# Autodesk Inventor assembly: Assembly3
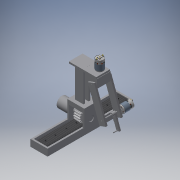
[picture p0: Inventor's stored thumbnail of the model, 180x180]
Saved by Autodesk Inventor 2019.4 (Build 234330000, 330)
## iProperties
Created: 2020-04-15
Part Number: Assembly3
Document SubType Name: Assembly
Designer: Niran
Author: Niran
## iProperties of the stored document S.gear.ipt
Created: 2020-04-14
Part Number: S.gear
Material: Generic
Document SubType Name: Modeling
Designer: Darugar
Density: 1 g/cm^3
Appearance: Default
Author: Darugar
Sending System: Autodesk Inventor 2020
## iProperties of the stored document S.motor.ipt
Created: 2020-04-14
Part Number: S.motor
Material: Generic
Document SubType Name: Modeling
Designer: Darugar
Density: 1 g/cm^3
Appearance: Default
Author: Darugar
Sending System: Autodesk Inventor 2020
## iProperties of the stored document S.Platform.ipt
Created: 2020-04-14
Part Number: S.Platform
Material: Generic
Document SubType Name: Modeling
Designer: Darugar
Density: 1 g/cm^3
Appearance: Default
Author: Darugar
Sending System: Autodesk Inventor 2020
## iProperties of the stored document s.Strikrt.ipt
Created: 2020-04-14
Part Number: s.Strikrt
Material: Generic
Document SubType Name: Modeling
Designer: Darugar
Density: 1 g/cm^3
Appearance: Default
Author: Darugar
Sending System: Autodesk Inventor 2020
## iProperties of the stored document S.rack.ipt
Created: 2020-04-14
Part Number: S.rack
Material: Generic
Document SubType Name: Modeling
Designer: Darugar
Density: 1 g/cm^3
Appearance: Default
Author: Darugar
Sending System: Autodesk Inventor 2020
## iProperties of the stored document S.hollow box.ipt
Created: 2020-04-13
Part Number: S.hollow box
Material: Generic
Document SubType Name: Modeling
Designer: Darugar
Density: 1 g/cm^3
Appearance: Default
Author: Darugar
Sending System: Autodesk Inventor 2020
## Documents named in this file (20)
- **C:\Users\Niran\Desktop\S.Carrom_bot\Assembly3.iam*LocalDocs*xDrle05f4Rw1buugfIqzzd3tlMb*S.gear.ipt
- **C:\Users\Niran\Desktop\S.Carrom_bot\Assembly3.iam*LocalDocs*x122kn5ufNzxlefwdNu51dwe40f*S.motor.ipt
- **C:\Users\Niran\Desktop\S.Carrom_bot\Assembly3.iam*LocalDocs*x0acgfz2z0tlie3kiGyxgdtb3Ig*S.Platform.ipt
- **C:\Users\Niran\Desktop\S.Carrom_bot\Assembly3.iam*LocalDocs*xOnqyxwphSiaaenkcZqvwvmabYh*s.Strikrt.ipt
- **C:\Users\Niran\Desktop\S.Carrom_bot\Assembly3.iam*LocalDocs*xMjvgupfc2g05uukt4i5agsne0h*S.rack.ipt
- **C:\Users\Niran\Desktop\S.Carrom_bot\Assembly3.iam*LocalDocs*xZqkpyfp0KfdfunouZc1cgw1dQb*S.hollow box.ipt
- C:\Users\Niran\Desktop\S.Carrom_bot\Assembly3.iam
- C:\Users\Niran\Desktop\S.Carrom_bot\S.Part1143.ipt
- C:\Users\Niran\Desktop\S.Carrom_bot\DC Motor.ipt
- C:\Users\Niran\Desktop\sketch_jan26a\Canon parts\Part36.ipt
- C:\Users\Niran\Desktop\S.Carrom_bot\Part59.ipt
- C:\Users\Niran\Desktop\S.Carrom_bot\Part13.ipt
- C:\Users\Niran\Desktop\S.Carrom_bot\Part14.ipt
- C:\Users\Niran\Desktop\sketch_jan26a\Canon parts\DC Motor.ipt
- C:\Users\Niran\Desktop\S.Carrom_bot\S.hollow box.ipt
- C:\Users\Niran\Desktop\S.Carrom_bot\S.rack.ipt
- C:\Users\Niran\Desktop\S.Carrom_bot\S.Platform.ipt
- C:\Users\Niran\Desktop\S.Carrom_bot\S.motor.ipt
- C:\Users\Niran\Desktop\S.Carrom_bot\S.gear.ipt
- C:\Users\Niran\Desktop\S.Carrom_bot\s.Strikrt.ipt
## Components (16 placed, 12 different names)
1. S.hollow box:1 — Rotational:1, Rotational:2
2. S.rack:1 — Rotational:1
3. S.Platform:1 — Rotational:2, Rotational:3, Rigid:3
4. S.motor:1 — Rotational:3, Rigid:1
5. S.gear:1 — Rigid:1
6. S.Part1143:1 — Rigid:2, Rigid:3
7. S.Part1143:2 — Rigid:2, Rigid:4, Rotational:4, Rotational:5
8. DC Motor:1 — Rigid:4
9. Part59:1 — Rotational:4
10. Part13:1 — Rotational:5, Rotational:6, Rotational:7
11. Part14:1 — Rotational:6, Rotational:8
12. Part14:2 — Rotational:7
13. Part36:1 — Rotational:8, Rotational:9, Rotational:10, Rigid:5
14. Part36:3 — Rotational:10
15. s.Strikrt:1 — Rotational:9
16. DC Motor:2 — Rigid:5
## Relationships (15: RevoluteJoint 10, WeldJoint 5)
- Rotational:1 [RevoluteJoint]: S.hollow box:1 ↔ S.rack:1
- Rotational:2 [RevoluteJoint]: S.hollow box:1 ↔ S.Platform:1
- Rotational:3 [RevoluteJoint]: S.Platform:1 ↔ S.motor:1
- Rigid:1 [WeldJoint] (-15 mm): S.motor:1 ↔ S.gear:1
- Rigid:2 [WeldJoint]: S.Part1143:1 ↔ S.Part1143:2
- Rigid:3 [WeldJoint]: S.Platform:1 ↔ S.Part1143:1
- Rigid:4 [WeldJoint] (10 mm): S.Part1143:2 ↔ DC Motor:1
- Rotational:4 [RevoluteJoint] (10 mm): S.Part1143:2 ↔ Part59:1
- Rotational:5 [RevoluteJoint]: S.Part1143:2 ↔ Part13:1
- Rotational:6 [RevoluteJoint]: Part13:1 ↔ Part14:1
- Rotational:7 [RevoluteJoint]: Part13:1 ↔ Part14:2
- Rotational:8 [RevoluteJoint] (-30 mm): Part14:1 ↔ Part36:1
- Rotational:9 [RevoluteJoint]: Part36:1 ↔ s.Strikrt:1
- Rotational:10 [RevoluteJoint] (60 mm): Part36:1 ↔ Part36:3
- Rigid:5 [WeldJoint] (4 mm): Part36:1 ↔ DC Motor:2
